# Autodesk Inventor assembly: Assembly1
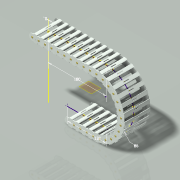
[picture p0: Inventor's stored thumbnail of the model, 180x180]
Saved by Autodesk Inventor 2015 (Build 190159000, 159)
## iProperties
Created: 2015-06-01
Part Number: Assembly1
Document SubType Name: Assembly
Designer: cad16
Author: cad16
## Documents named in this file (3)
- D:\rantai1\Assembly1.iam
- D:\rantai1\path.ipt
- D:\rantai1\Part1.ipt
## Components (28 placed, 2 different names)
1. path:1 — Mate:1, Mate:2, Mate:4, Mate:6, Mate:7
2. Part1:1 — Mate:7, Angle:3
3. Part1:2
4. Part1:3
5. Part1:4
6. Part1:5
7. Part1:6
8. Part1:7
9. Part1:8
10. Part1:9
11. Part1:10
12. Part1:11
13. Part1:12
14. Part1:13
15. Part1:14
16. Part1:15
17. Part1:16
18. Part1:17
19. Part1:18
20. Part1:19
21. Part1:20
22. Part1:21
23. Part1:22
24. Part1:23
25. Part1:24
26. Part1:25
27. Part1:26
28. Part1:27
## Component patterns: (27 elements, first: Part1:1)
## Relationships (7: Mate 5, Angle 2)
- Mate:1: path:1
- Mate:2: path:1
- Mate:4: path:1
- Angle:2 (0 deg)
- Mate:6: path:1
- Mate:7: path:1 ↔ Part1:1
- Angle:3 (0 deg): Part1:1
